# Autodesk Inventor assembly: Drawer
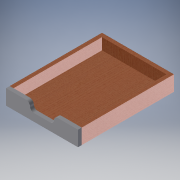
[picture p0: Inventor's stored thumbnail of the model, 180x180]
Saved by Autodesk Inventor 2016 (Build 200138000, 138)
## iProperties
Created: 2017-10-31
Part Number: Drawer
Document SubType Name: Assembly
Designer: mathaetaes
Author: mathaetaes
## Documents named in this file (6)
- E:\Projects\3D Printer\printer projects\My Designs\Bar Cabinet\Drawer.iam
- E:\Projects\3D Printer\printer projects\My Designs\Bar Cabinet\Drawer sides.ipt
- E:\Projects\3D Printer\printer projects\My Designs\Bar Cabinet\Drawer ends.ipt
- E:\Projects\3D Printer\printer projects\My Designs\Bar Cabinet\Drawer Side Supports.ipt
- E:\Projects\3D Printer\printer projects\My Designs\Bar Cabinet\Drawer bottom.ipt
- E:\Projects\3D Printer\printer projects\My Designs\Bar Cabinet\Drawer Front.ipt
## Components (7 placed, 5 different names)
1. Drawer sides:1 — Flush:1, Flush:2, Mate:1, Flush:5, Mate:3, Flush:9, Mate:7, Mate:9, Flush:11, Flush:12, Mate:11
2. Drawer sides:2 — Flush:1, Flush:2, Mate:1, Flush:6, Flush:8, Flush:10, Mate:6
3. Drawer ends:2 — Flush:5, Flush:6, Flush:8, Mate:3, Mate:4, Mate:5, Mate:8
4. Drawer Side Supports:1 — Flush:10, Mate:4, Mate:7, Mate:10
5. Drawer Side Supports:2 — Flush:9, Mate:5, Mate:6
6. Drawer bottom:1 — Mate:8, Mate:9, Mate:10
7. Drawer Front:1 — Flush:11, Flush:12, Mate:11
## Relationships (19: Mate 10, Flush 9)
- Flush:1: Drawer sides:1 ↔ Drawer sides:2
- Flush:2: Drawer sides:1 ↔ Drawer sides:2
- Mate:1 (323.85 mm): Drawer sides:1 ↔ Drawer sides:2
- Flush:5: Drawer sides:1 ↔ Drawer ends:2
- Flush:6: Drawer sides:2 ↔ Drawer ends:2
- Flush:8: Drawer sides:2 ↔ Drawer ends:2
- Mate:3: Drawer sides:1 ↔ Drawer ends:2
- Flush:9: Drawer sides:1 ↔ Drawer Side Supports:2
- Flush:10: Drawer sides:2 ↔ Drawer Side Supports:1
- Mate:4: Drawer ends:2 ↔ Drawer Side Supports:1
- Mate:5: Drawer ends:2 ↔ Drawer Side Supports:2
- Mate:6: Drawer sides:2 ↔ Drawer Side Supports:2
- Mate:7: Drawer sides:1 ↔ Drawer Side Supports:1
- Mate:8: Drawer ends:2 ↔ Drawer bottom:1
- Mate:9: Drawer sides:1 ↔ Drawer bottom:1
- Mate:10: Drawer Side Supports:1 ↔ Drawer bottom:1
- Flush:11: Drawer sides:1 ↔ Drawer Front:1
- Flush:12: Drawer sides:1 ↔ Drawer Front:1
- Mate:11: Drawer sides:1 ↔ Drawer Front:1
